# Autodesk Inventor assembly: LED housing Assembly
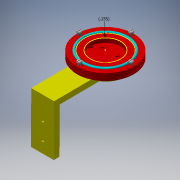
[picture p0: Inventor's stored thumbnail of the model, 180x180]
Saved by Autodesk Inventor 2016 (Build 200138000, 138)
## iProperties
Created: 2017-09-28
Part Number: LED housing Assembly
Document SubType Name: Assembly
Designer: Student
Author: Student
## Documents named in this file (6)
- C:\Users\Student\Documents\Derek Code and Projects\Autodesk\LED housing Assembly.iam
- C:\Users\Student\Documents\Derek Code and Projects\Autodesk\Acrylic Lens.ipt
- C:\Users\Student\Documents\Derek Code and Projects\Autodesk\LED holder 2.ipt
- C:\Users\Student\Documents\Derek Code and Projects\Autodesk\O-ring for LED Acrylic.ipt
- C:\Users\Student\Documents\Inventor\Content Center Files\R2016\en-US\BS 4183(7)\BS 4183 - M2.5 x 5(2) III.ipt
- C:\Users\Student\Documents\Derek Code and Projects\Autodesk\LED Hinge.ipt
## Components (14 placed, 5 different names)
1. Acrylic Lens:1 — Mate:1, Mate:2, Insert:5, Insert:6, Insert:7, Insert:8
2. LED holder 2:1 — Mate:1, Mate:2, Mate:3, Mate:4
3. O-ring for LED Acrylic:1 — Mate:3
4. BS 4183 Slotted Pan Head Machine Screw - Metric M2.5 x 5:5 — Insert:5
5. BS 4183 Slotted Pan Head Machine Screw - Metric M2.5 x 5:6 — Insert:6
6. BS 4183 Slotted Pan Head Machine Screw - Metric M2.5 x 5:7 — Insert:7
7. BS 4183 Slotted Pan Head Machine Screw - Metric M2.5 x 5:8 — Insert:8
8. LED Hinge:1 — Mate:4, Insert:9, Insert:10, Insert:11, Insert:12, Insert:13, Insert:14
9. BS 4183 Slotted Pan Head Machine Screw - Metric M2.5 x 5:9 — Insert:9
10. BS 4183 Slotted Pan Head Machine Screw - Metric M2.5 x 5:10 — Insert:10
11. BS 4183 Slotted Pan Head Machine Screw - Metric M2.5 x 5:11 — Insert:11
12. BS 4183 Slotted Pan Head Machine Screw - Metric M2.5 x 5:12 — Insert:12
13. BS 4183 Slotted Pan Head Machine Screw - Metric M2.5 x 5:13 — Insert:13
14. BS 4183 Slotted Pan Head Machine Screw - Metric M2.5 x 5:14 — Insert:14
## Relationships (14: Insert 10, Mate 4)
- Mate:1: Acrylic Lens:1 ↔ LED holder 2:1
- Mate:2: Acrylic Lens:1 ↔ LED holder 2:1
- Mate:3: LED holder 2:1 ↔ O-ring for LED Acrylic:1
- Insert:5: Acrylic Lens:1 ↔ BS 4183 Slotted Pan Head Machine Screw - Metric M2.5 x 5:5
- Insert:6: Acrylic Lens:1 ↔ BS 4183 Slotted Pan Head Machine Screw - Metric M2.5 x 5:6
- Insert:7: Acrylic Lens:1 ↔ BS 4183 Slotted Pan Head Machine Screw - Metric M2.5 x 5:7
- Insert:8: Acrylic Lens:1 ↔ BS 4183 Slotted Pan Head Machine Screw - Metric M2.5 x 5:8
- Mate:4: LED holder 2:1 ↔ LED Hinge:1
- Insert:9: LED Hinge:1 ↔ BS 4183 Slotted Pan Head Machine Screw - Metric M2.5 x 5:9
- Insert:10: LED Hinge:1 ↔ BS 4183 Slotted Pan Head Machine Screw - Metric M2.5 x 5:10
- Insert:11: LED Hinge:1 ↔ BS 4183 Slotted Pan Head Machine Screw - Metric M2.5 x 5:11
- Insert:12: LED Hinge:1 ↔ BS 4183 Slotted Pan Head Machine Screw - Metric M2.5 x 5:12
- Insert:13: LED Hinge:1 ↔ BS 4183 Slotted Pan Head Machine Screw - Metric M2.5 x 5:13
- Insert:14: LED Hinge:1 ↔ BS 4183 Slotted Pan Head Machine Screw - Metric M2.5 x 5:14
